# Autodesk Inventor assembly: Assieme 1 - Trasporto
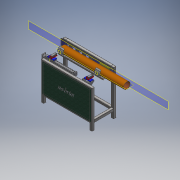
[picture p0: Inventor's stored thumbnail of the model, 180x180]
Saved by Autodesk Inventor 2018 (Build 220112000, 112)
## iProperties
Created: 2020-05-30
Part Number: Assieme 1 - Trasporto
Material: Generico
Document SubType Name: Weldment
Designer: Francesco
Weld Material: Welded Aluminum-6061
Author: Francesco
## Documents named in this file (11)
- C:\Users\Francesco\no-brim\Meccanica\Progetto Inventor no-brim\Assiemi\Assieme 1 - Trasporto.iam
- C:\Users\Francesco\no-brim\Meccanica\Progetto Inventor no-brim\Assiemi\Telaio - Trasporto.iam
- C:\Users\Francesco\no-brim\Meccanica\Progetto Inventor no-brim\Assiemi\Rulliera - Trasporto.iam
- C:\Users\Francesco\no-brim\Meccanica\Progetto Inventor no-brim\Parti\Lamiera riferimento.ipt
- C:\Users\Francesco\no-brim\Meccanica\Progetto Inventor no-brim\Parti\Spessore plastica.ipt
- C:\Users\Francesco\no-brim\Meccanica\Progetto Inventor no-brim\Parti\Tubo.ipt
- C:\Users\Francesco\no-brim\Meccanica\Progetto Inventor no-brim\Assiemi\Pistoni pinza - Trasporto.iam
- C:\Users\Francesco\no-brim\Meccanica\Progetto Inventor no-brim\Parti\Asse lineare corsa 300 mm\Assieme asse lineare corsa 300 mm.iam
- C:\Users\Francesco\no-brim\Meccanica\Progetto Inventor no-brim\Parti\Piastra sostegno asse.ipt
- C:\Users\Francesco\no-brim\Meccanica\Progetto Inventor no-brim\Parti\Lamiera logo no-brim.ipt
- C:\Users\Francesco\no-brim\Meccanica\Progetto Inventor no-brim\Assiemi\Supporto saldato pistone 2 - Trasporto.iam
## Components (15 placed, 10 different names)
1. Telaio - Trasporto:1 [sub-assembly] — Coincidente:1, Coincidente:2, Coincidente:3, Coincidente:4, Coincidente:5, Coincidente:6, Coincidente:7, Coincidente:8, Coincidente:9, Coincidente:10, Coincidente:11, Angolo:1, Angolo:3, Coincidente:16, Angolo:4, Coincidente:20, Allineato:11, Coincidente:21, Coincidente:23, Allineato:14, Allineato:15, Coincidente:24
2. Rulliera - Trasporto:1 [sub-assembly] — Coincidente:1, Coincidente:5
3. Rulliera - Trasporto:2 [sub-assembly] — Coincidente:3, Coincidente:8
4. Rulliera - Trasporto:3 [sub-assembly] — Coincidente:2, Coincidente:6, Allineato:1
5. Rulliera - Trasporto:4 [sub-assembly] — Coincidente:4, Coincidente:7
6. Lamiera riferimento:1 — Coincidente:9, Coincidente:10, Coincidente:11, Coincidente:12, Coincidente:13, Coincidente:14, Coincidente:15, Allineato:6, Allineato:10
7. Spessore plastica:1 — Coincidente:12, Coincidente:13, Coincidente:14, Allineato:5
8. Tubo:1 — Angolo:1, Allineato:2, Angolo:2, Tangente:1, Coincidente:17, Allineato:10
9. Pistoni pinza - Trasporto:1 [sub-assembly] — Angolo:3, Coincidente:16, Coincidente:17, Allineato:3, Allineato:4, Allineato:6, Coincidente:19, Allineato:8, Allineato:9
10. Pistoni pinza - Trasporto:2 [sub-assembly] — Allineato:3, Allineato:4, Allineato:5, Coincidente:25, Coincidente:26
11. Assieme asse lineare corsa 300 mm:1 [sub-assembly] — Angolo:4, Coincidente:19, Allineato:7, Allineato:9
12. Piastra sostegno asse:1 — Coincidente:20, Allineato:11, Coincidente:21, Allineato:12, Allineato:13, Coincidente:22
13. Piastra sostegno asse:2 — Allineato:12, Allineato:13, Coincidente:22
14. Lamiera logo no-brim:1 — Coincidente:23, Allineato:14, Allineato:15
15. Supporto saldato pistone 2:1 [sub-assembly] — Coincidente:24, Coincidente:25, Coincidente:26
## Relationships (45: Mate 25, Flush 15, Angle 4, Tangent 1)
- Coincidente:1 [Mate]: Telaio - Trasporto:1 ↔ Rulliera - Trasporto:1
- Coincidente:2 [Mate]: Telaio - Trasporto:1 ↔ Rulliera - Trasporto:3
- Coincidente:3 [Mate]: Telaio - Trasporto:1 ↔ Rulliera - Trasporto:2
- Coincidente:4 [Mate]: Telaio - Trasporto:1 ↔ Rulliera - Trasporto:4
- Coincidente:5 [Mate]: Telaio - Trasporto:1 ↔ Rulliera - Trasporto:1
- Coincidente:6 [Mate]: Telaio - Trasporto:1 ↔ Rulliera - Trasporto:3
- Coincidente:7 [Mate]: Telaio - Trasporto:1 ↔ Rulliera - Trasporto:4
- Coincidente:8 [Mate]: Telaio - Trasporto:1 ↔ Rulliera - Trasporto:2
- Coincidente:9 [Mate]: Telaio - Trasporto:1 ↔ Lamiera riferimento:1
- Coincidente:10 [Mate]: Telaio - Trasporto:1 ↔ Lamiera riferimento:1
- Coincidente:11 [Mate] (5 mm): Telaio - Trasporto:1 ↔ Lamiera riferimento:1
- Coincidente:12 [Mate]: Lamiera riferimento:1 ↔ Spessore plastica:1
- Coincidente:13 [Mate]: Lamiera riferimento:1 ↔ Spessore plastica:1
- Coincidente:14 [Mate]: Lamiera riferimento:1 ↔ Spessore plastica:1
- Angolo:1 [Angle] (0 deg): Telaio - Trasporto:1 ↔ Tubo:1
- Allineato:1 [Flush] (13.5 mm): Rulliera - Trasporto:3
- Allineato:2 [Flush]: Tubo:1
- Angolo:2 [Angle] (0 deg): Tubo:1
- Tangente:1: Tubo:1
- Coincidente:15 [Mate]: Lamiera riferimento:1
- Angolo:3 [Angle] (0 deg): Telaio - Trasporto:1 ↔ Pistoni pinza - Trasporto:1
- Coincidente:16 [Mate] (22 mm): Telaio - Trasporto:1 ↔ Pistoni pinza - Trasporto:1
- Coincidente:17 [Mate]: Tubo:1 ↔ Pistoni pinza - Trasporto:1
- Allineato:3 [Flush]: Pistoni pinza - Trasporto:1 ↔ Pistoni pinza - Trasporto:2
- Allineato:4 [Flush]: Pistoni pinza - Trasporto:1 ↔ Pistoni pinza - Trasporto:2
- Allineato:5 [Flush]: Spessore plastica:1 ↔ Pistoni pinza - Trasporto:2
- Allineato:6 [Flush]: Lamiera riferimento:1 ↔ Pistoni pinza - Trasporto:1
- Angolo:4 [Angle] (0 deg): Telaio - Trasporto:1 ↔ Assieme asse lineare corsa 300 mm:1
- Coincidente:19 [Mate] (8 mm): Pistoni pinza - Trasporto:1 ↔ Assieme asse lineare corsa 300 mm:1
- Allineato:7 [Flush] (-55 mm): Assieme asse lineare corsa 300 mm:1
- Allineato:8 [Flush]: Pistoni pinza - Trasporto:1
- Allineato:9 [Flush]: Pistoni pinza - Trasporto:1 ↔ Assieme asse lineare corsa 300 mm:1
- Allineato:10 [Flush] (-250 mm): Lamiera riferimento:1 ↔ Tubo:1
- Coincidente:20 [Mate]: Telaio - Trasporto:1 ↔ Piastra sostegno asse:1
- Allineato:11 [Flush] (5 mm): Telaio - Trasporto:1 ↔ Piastra sostegno asse:1
- Coincidente:21 [Mate] (50 mm): Telaio - Trasporto:1 ↔ Piastra sostegno asse:1
- Allineato:12 [Flush]: Piastra sostegno asse:1 ↔ Piastra sostegno asse:2
- Allineato:13 [Flush]: Piastra sostegno asse:1 ↔ Piastra sostegno asse:2
- Coincidente:22 [Mate] (200 mm): Piastra sostegno asse:1 ↔ Piastra sostegno asse:2
- Coincidente:23 [Mate]: Telaio - Trasporto:1 ↔ Lamiera logo no-brim:1
- Allineato:14 [Flush] (17.5 mm): Telaio - Trasporto:1 ↔ Lamiera logo no-brim:1
- Allineato:15 [Flush] (17.5 mm): Telaio - Trasporto:1 ↔ Lamiera logo no-brim:1
- Coincidente:24 [Mate]: Telaio - Trasporto:1 ↔ Supporto saldato pistone 2:1
- Coincidente:25 [Mate]: Pistoni pinza - Trasporto:2 ↔ Supporto saldato pistone 2:1
- Coincidente:26 [Mate]: Pistoni pinza - Trasporto:2 ↔ Supporto saldato pistone 2:1
